# Autodesk Inventor assembly: Full Prober assembly
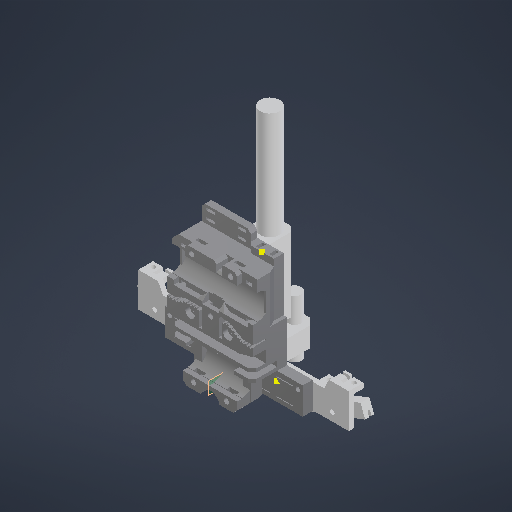
[picture p0: Inventor's stored thumbnail of the model, 512x512]
Saved by Autodesk Inventor 2026 (Build 300175050, 175E)
## iProperties
Created: 2025-07-01
Part Number: Full Prober assembly
Document SubType Name: Assembly
Designer: Tobymegacat
Author: Tobymegacat
## Documents named in this file (10)
- C:\Users\herve\OneDrive\桌面\NIST\Inventor\Full Prober assembly.iam
- C:\Users\herve\Downloads\x-carriage(R2)\x-carriage(R2)\x-carriage(R2).ipt
- C:\Users\herve\OneDrive\桌面\NIST\Inventor\dummy microscope.ipt
- C:\Users\herve\OneDrive\桌面\NIST\Inventor\dummy Z axis sensor.ipt
- C:\Users\herve\OneDrive\桌面\NIST\Inventor\microscope mount.ipt
- C:\Users\herve\OneDrive\桌面\NIST\Inventor\Assembly1.iam
- C:\Users\herve\OneDrive\桌面\NIST\Inventor\probe mount 1 side.ipt
- C:\Users\herve\OneDrive\桌面\NIST\Inventor\probe mount 1 side_MIR.ipt
- C:\Users\herve\OneDrive\桌面\NIST\Inventor\Z axis collar.ipt
- C:\Users\herve\OneDrive\桌面\NIST\Inventor\Assembly1_MIR.iam
## Components (9 placed, 9 different names)
1. x-carriage(R2):1 — Flush:1, Rigid:2, Flush:2, Rotational:2, Rigid:3, Rotational:4
2. dummy microscope:1 — Rigid:1, Rigid:4
3. dummy Z axis sensor:1 — Rigid:5
4. microscope mount:1 — Flush:1, Rigid:1, Rigid:2
5. Assembly1:1 [sub-assembly] — Rotational:1
6. probe mount 1 side:1 — Flush:2, Rotational:1, Rotational:2, Rigid:3
7. probe mount 1 side_MIR:1 — Rotational:4, Rotational:5
8. Z axis collar:1 — Rigid:4, Rigid:5
9. Assembly1_MIR:1 [sub-assembly] — Rotational:5
## Relationships (11: WeldJoint 5, RevoluteJoint 4, Flush 2)
- Flush:1: x-carriage(R2):1 ↔ microscope mount:1
- Rigid:1 [WeldJoint] (-30 mm): dummy microscope:1 ↔ microscope mount:1
- Rigid:2 [WeldJoint]: x-carriage(R2):1 ↔ microscope mount:1
- Flush:2: x-carriage(R2):1 ↔ probe mount 1 side:1
- Rotational:1 [RevoluteJoint]: Assembly1:1 ↔ probe mount 1 side:1
- Rotational:2 [RevoluteJoint]: x-carriage(R2):1 ↔ probe mount 1 side:1
- Rigid:3 [WeldJoint]: x-carriage(R2):1 ↔ probe mount 1 side:1
- Rotational:4 [RevoluteJoint]: x-carriage(R2):1 ↔ probe mount 1 side_MIR:1
- Rigid:4 [WeldJoint] (-8 mm): dummy microscope:1 ↔ Z axis collar:1
- Rigid:5 [WeldJoint] (8 mm): dummy Z axis sensor:1 ↔ Z axis collar:1
- Rotational:5 [RevoluteJoint]: probe mount 1 side_MIR:1 ↔ Assembly1_MIR:1
